# Autodesk Inventor assembly: splashAssembly
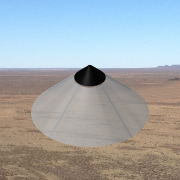
[picture p0: Inventor's stored thumbnail of the model, 180x180]
Saved by Autodesk Inventor 2013 SP2 (Build 170200200, 200)
## iProperties
Created: 2013-06-11
Part Number: splashAssembly
Document SubType Name: Assembly
Designer: Dave
Author: Dave
## Documents named in this file (4)
- C:\Users\Dave\Desktop\HERA\splashAssembly.iam
- C:\Users\Dave\Desktop\HERA\splash_base.ipt
- C:\Users\Dave\Desktop\HERA\splash_shortPVC.ipt
- C:\Users\Dave\Desktop\HERA\splash_top.ipt
## Components (6 placed, 3 different names)
1. splash_base:1 — Insert:1
2. splash_top:1 — Insert:1
3. splash_shortPVC:1
4. splash_shortPVC:2
5. splash_shortPVC:3
6. splash_shortPVC:4
## Component patterns: (4 elements, first: splash_shortPVC:1)
## Relationships (1: Insert 1)
- Insert:1 (12.7 mm): splash_base:1 ↔ splash_top:1
